# Autodesk Inventor assembly: Camera mount assembly
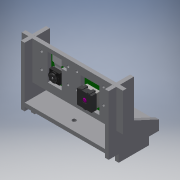
[picture p0: Inventor's stored thumbnail of the model, 180x180]
Saved by Autodesk Inventor 2018 (Build 220112000, 112)
## iProperties
Created: 2018-05-02
Part Number: Camera mount assembly
Document SubType Name: Assembly
Designer: Ajith Thomas
Author: Ajith Thomas
## Documents named in this file (6)
- C:\Users\Ajith Thomas\Dropbox\Gas_Sensing_Robot\FumeBot-Design\Camera mount assembly.iam
- C:\Users\Ajith Thomas\Dropbox\Gas_Sensing_Robot\FumeBot-Design\Sensors and Boards\Raspberry Pi Camera\RasPi_Camera.iam
- C:\Users\Ajith Thomas\Dropbox\Gas_Sensing_Robot\FumeBot-Design\Sensors and Boards\Lepton 3 Thermal Camera\Lepton 3 thermal camera.iam
- C:\Users\Ajith Thomas\Dropbox\Gas_Sensing_Robot\FumeBot-Design\Camera bracket.ipt
- C:\Users\Ajith Thomas\Dropbox\Gas_Sensing_Robot\FumeBot-Design\Camera bracket raiser.ipt
- C:\Users\Ajith Thomas\Dropbox\Gas_Sensing_Robot\FumeBot-Design\Camera cross bar.ipt
## Components (6 placed, 5 different names)
1. RasPi_Camera:1 [sub-assembly] — Distance RPI and Thermal, Flush:1, Flush:2, Flush:3
2. Lepton 3 thermal camera:1 [sub-assembly] — Distance RPI and Thermal, Flush:1, Flush:2
3. Camera bracket:1 — Flush:3, Flush:4
4. Camera bracket raiser:1 — Flush:4, Flush:5
5. Camera cross bar:1 — Flush:5, Mate:2, Flush:6, Mate:3
6. Camera bracket raiser:2 — Mate:2, Flush:6, Mate:3
## Relationships (9: Flush 6, Mate 3)
- Distance RPI and Thermal [Mate] (3 mm): RasPi_Camera:1 ↔ Lepton 3 thermal camera:1
- Flush:1: RasPi_Camera:1 ↔ Lepton 3 thermal camera:1
- Flush:2: RasPi_Camera:1 ↔ Lepton 3 thermal camera:1
- Flush:3: RasPi_Camera:1 ↔ Camera bracket:1
- Flush:4: Camera bracket:1 ↔ Camera bracket raiser:1
- Flush:5: Camera bracket raiser:1 ↔ Camera cross bar:1
- Mate:2: Camera cross bar:1 ↔ Camera bracket raiser:2
- Flush:6: Camera cross bar:1 ↔ Camera bracket raiser:2
- Mate:3: Camera cross bar:1 ↔ Camera bracket raiser:2
